# Autodesk Inventor assembly: BearingBlockAssembly
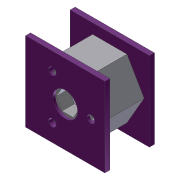
[picture p0: Inventor's stored thumbnail of the model, 180x180]
Saved by Autodesk Inventor 2012 (Build 160160000, 160)
## iProperties
Created: 2012-11-17
Part Number: BearingBlockAssembly
Document SubType Name: Assembly
Designer: JesseK
Author: JesseK
## Documents named in this file (4)
- Z:\UserData\Documents\Inventor\team1885frc\Robot2013\DriveTrainProto\BearingBlockAssembly.iam
- Z:\UserData\Documents\Inventor\team1885frc\Robot2013\DriveTrainProto\BearingBlock.ipt
- Z:\UserData\Documents\Inventor\team1885frc\Robot2013\DriveTrainProto\BearingRetainerPlate.ipt
- Z:\UserData\Documents\Inventor\team1885frc\Hardware\Bearings\500id_1.125od_hex_flange_bearing.ipt
## Components (5 placed, 3 different names)
1. BearingBlock:1 — Mate:1, Mate:2, Mate:3, Mate:4, Mate:5, Mate:6, Mate:7, Mate:8, Mate:9, Mate:10
2. BearingRetainerPlate:1 — Mate:1, Mate:2, Mate:3
3. BearingRetainerPlate:2 — Mate:4, Mate:5, Mate:6
4. 500id_1.125od_hex_flange_bearing:1 — Mate:9, Mate:10
5. 500id_1.125od_hex_flange_bearing:2 — Mate:7, Mate:8
## Relationships (10: Mate 10)
- Mate:1: BearingBlock:1 ↔ BearingRetainerPlate:1
- Mate:2: BearingBlock:1 ↔ BearingRetainerPlate:1
- Mate:3: BearingBlock:1 ↔ BearingRetainerPlate:1
- Mate:4: BearingBlock:1 ↔ BearingRetainerPlate:2
- Mate:5: BearingBlock:1 ↔ BearingRetainerPlate:2
- Mate:6: BearingBlock:1 ↔ BearingRetainerPlate:2
- Mate:7: BearingBlock:1 ↔ 500id_1.125od_hex_flange_bearing:2
- Mate:8: BearingBlock:1 ↔ 500id_1.125od_hex_flange_bearing:2
- Mate:9: BearingBlock:1 ↔ 500id_1.125od_hex_flange_bearing:1
- Mate:10: BearingBlock:1 ↔ 500id_1.125od_hex_flange_bearing:1
